# Autodesk Inventor assembly: main
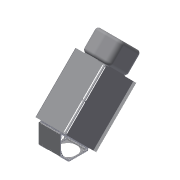
[picture p0: Inventor's stored thumbnail of the model, 180x180]
Saved by Autodesk Inventor 2014 SP1 (Build 180222100, 222)
## iProperties
Created: 2015-02-04
Part Number: main
Document SubType Name: Assembly
Designer: Simen
Author: Simen
## Documents named in this file (8)
- C:\Users\Simen\Documents\git\Eit\skjellet\main.iam
- C:\Users\Simen\Documents\git\Eit\skjellet\base.iam
- C:\Users\Simen\Documents\git\Eit\skjellet\skellett.iam
- C:\Users\Simen\Documents\git\Eit\skjellet\Head.iam
- C:\Users\Simen\Documents\git\Eit\skjellet\Side104x700.ipt
- C:\Users\Simen\Documents\git\Eit\skjellet\side500x1040.ipt
- C:\Users\Simen\Documents\git\Eit\skjellet\side350x390.ipt
- C:\Users\Simen\Documents\git\Eit\skjellet\side350x390_hull.ipt
## Components (9 placed, 7 different names)
1. base:1 [sub-assembly] — Mate:1, Flush:1, Mate:3
2. skellett:1 [sub-assembly] — Mate:1, Flush:1, Mate:3, Flush:2, Mate:4, Flush:3, Flush:4, Flush:5, Flush:6, Flush:7, Flush:8, Flush:9, Flush:10, Flush:13
3. Head:1 [sub-assembly] — Flush:2, Mate:4, Flush:11, Flush:12, Flush:13, Flush:14, Flush:15
4. Side104x700:1 — Flush:3, Flush:4
5. Side104x700:2 — Flush:5, Flush:6
6. side500x1040:1 — Flush:7, Flush:8
7. side500x1040:2 — Flush:9, Flush:10
8. side350x390:1 — Flush:11, Flush:12
9. side350x390_hull:1 — Flush:14, Flush:15
## Relationships (18: Flush 15, Mate 3)
- Mate:1: base:1 ↔ skellett:1
- Flush:1: base:1 ↔ skellett:1
- Mate:3 (-100 mm): base:1 ↔ skellett:1
- Flush:2: skellett:1 ↔ Head:1
- Mate:4: skellett:1 ↔ Head:1
- Flush:3: skellett:1 ↔ Side104x700:1
- Flush:4: skellett:1 ↔ Side104x700:1
- Flush:5: skellett:1 ↔ Side104x700:2
- Flush:6: skellett:1 ↔ Side104x700:2
- Flush:7: skellett:1 ↔ side500x1040:1
- Flush:8: skellett:1 ↔ side500x1040:1
- Flush:9: skellett:1 ↔ side500x1040:2
- Flush:10: skellett:1 ↔ side500x1040:2
- Flush:11: Head:1 ↔ side350x390:1
- Flush:12: Head:1 ↔ side350x390:1
- Flush:13 (55 mm): skellett:1 ↔ Head:1
- Flush:14: Head:1 ↔ side350x390_hull:1
- Flush:15: Head:1 ↔ side350x390_hull:1
